# Autodesk Inventor assembly: Nut+Washer M8
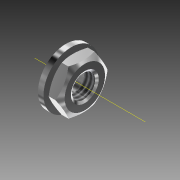
[picture p0: Inventor's stored thumbnail of the model, 180x180]
Saved by Autodesk Inventor 2013 (Build 170138000, 138)
## iProperties
Created: 2013-01-04
Part Number: Nut+Washer M8
Document SubType Name: Assembly
Designer: Nico
Author: Nico
## Documents named in this file (3)
- D:\Documents\Inventor\Coil winder\IAM files\Nut+Washer M8.iam
- D:\Documents\Inventor\Coil winder\IPT files\Washer M8.ipt
- D:\Documents\Inventor\Coil winder\IPT files\Half Nut M8.ipt
## Components (2 placed, 2 different names)
1. Washer M8:1 — Mate:1, Mate:2
2. Half Nut M8:1 — Mate:1, Mate:2
## Relationships (2: Mate 2)
- Mate:1: Washer M8:1 ↔ Half Nut M8:1
- Mate:2: Washer M8:1 ↔ Half Nut M8:1
